# Autodesk Inventor assembly: HbIndexFinger01ForChild_MIR
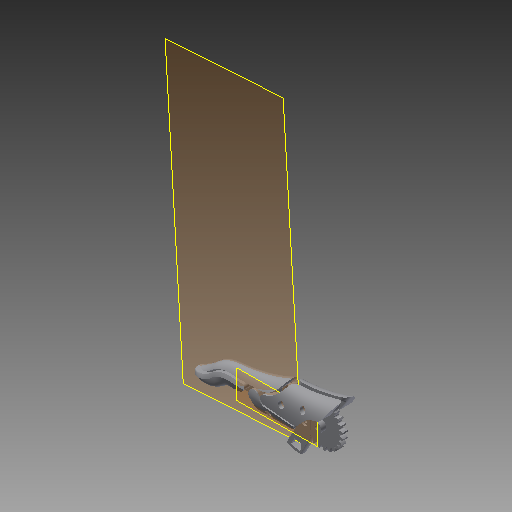
[picture p0: Inventor's stored thumbnail of the model, 512x512]
Saved by Autodesk Inventor 2017 (Build 210142000, 142)
## iProperties
Part Number: HbIndexFinger01ForChild_MIR
Material: 一般
Document SubType Name: Assembly
Designer: sktom
Author: sktom
## Documents named in this file (8)
- D:\OneDrive\CAD\MAJ\hackberry\HACKberry-hardware\3D_69%inlength\Inventor_right\HbHandForChild\HbIndexFinger01ForChild\HbIndexFinger01ForChild_MIR.iam
- D:\OneDrive\CAD\MAJ\hackberry\HACKberry-hardware\3D_69%inlength\Inventor_right\HbHandForChild\HbIndexFinger01ForChild\HbIndexInputLink02ForChild_MIR.ipt
- D:\OneDrive\CAD\MAJ\hackberry\HACKberry-hardware\3D_69%inlength\Inventor_right\HbHandForChild\HbIndexFinger01ForChild\HbIndexMiddle-DistalPhalanx02ForChild_MIR.ipt
- D:\OneDrive\CAD\MAJ\hackberry\HACKberry-hardware\3D_69%inlength\Inventor_right\HbHandForChild\HbIndexFinger01ForChild\HbIndexCouplerLink02ForChild_MIR.ipt
- D:\OneDrive\CAD\MAJ\hackberry\HACKberry-hardware\3D_69%inlength\Inventor_right\HbHandForChild\HbIndexFinger01ForChild\HbIndexCouplerLinkCover02ForChild_MIR.ipt
- D:\OneDrive\CAD\MAJ\hackberry\HACKberry-hardware\3D_69%inlength\Inventor_right\HbHandForChild\HbIndexFinger01ForChild\HbIndexProximalPhalanx03ForChild_MIR.ipt
- D:\OneDrive\CAD\MAJ\hackberry\HACKberry-hardware\3D_69%inlength\Inventor_right\HbHandForChild\HbIndexFinger01ForChild\HbIndexProximalPhalanxCover02ForChild_MIR.ipt
- D:\OneDrive\CAD\MAJ\hackberry\HACKberry-hardware\3D_69%inlength\Inventor_right\HbHandForChild\HbIndexFinger01ForChild\HbIndexReleaseLever02ForChild_MIR.ipt
## Components (7 placed, 7 different names)
1. HbIndexInputLink02ForChild_MIR:1 — 挿入:4, 円柱状:1
2. HbIndexMiddle-DistalPhalanx02ForChild_MIR:1 — 挿入:1, 挿入:5
3. HbIndexCouplerLink02ForChild_MIR:1 — 挿入:4, 挿入:1, 挿入:3, 挿入:2
4. HbIndexCouplerLinkCover02ForChild_MIR:1 — 挿入:3, 挿入:2
5. HbIndexProximalPhalanx03ForChild_MIR:1
6. HbIndexProximalPhalanxCover02ForChild_MIR:1 — 挿入:5, 挿入:8, 円柱状:1
7. HbIndexReleaseLever02ForChild_MIR:1 — 挿入:8
## Relationships (7: Insert 6, CylindricalJoint 1)
- 挿入:4 [Insert] (0.25 mm): HbIndexInputLink02ForChild_MIR:1 ↔ HbIndexCouplerLink02ForChild_MIR:1
- 挿入:1 [Insert] (0.4 mm): HbIndexMiddle-DistalPhalanx02ForChild_MIR:1 ↔ HbIndexCouplerLink02ForChild_MIR:1
- 挿入:3 [Insert]: HbIndexCouplerLink02ForChild_MIR:1 ↔ HbIndexCouplerLinkCover02ForChild_MIR:1
- 挿入:2 [Insert]: HbIndexCouplerLink02ForChild_MIR:1 ↔ HbIndexCouplerLinkCover02ForChild_MIR:1
- 挿入:5 [Insert] (0.4 mm): HbIndexMiddle-DistalPhalanx02ForChild_MIR:1 ↔ HbIndexProximalPhalanxCover02ForChild_MIR:1
- 挿入:8 [Insert] (0.2 mm): HbIndexProximalPhalanxCover02ForChild_MIR:1 ↔ HbIndexReleaseLever02ForChild_MIR:1
- 円柱状:1 [CylindricalJoint]: HbIndexInputLink02ForChild_MIR:1 ↔ HbIndexProximalPhalanxCover02ForChild_MIR:1
